# Autodesk Inventor assembly: Robot Assembly
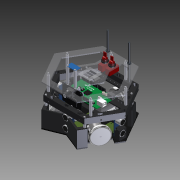
[picture p0: Inventor's stored thumbnail of the model, 180x180]
Saved by Autodesk Inventor 2015 (Build 190159000, 159)
## iProperties
Created: 2016-02-25
Part Number: Robot Assembly
Document SubType Name: Assembly
Designer: James Yelland
Author: James Yelland
## Documents named in this file (29)
- C:\Users\James Yelland\git\Design\Design\Models\Version 5\Robot Assembly.iam
- C:\Users\James Yelland\git\Design\Design\Models\Version 5\TSOP Array.ipt
- C:\Users\James Yelland\git\Design\Design\Models\Version 5\Bottom Plate.ipt
- C:\Users\James Yelland\git\Design\Design\Models\Version 5\Side Support.ipt
- C:\Users\James Yelland\git\Design\Design\Models\Version 5\Front Support.ipt
- C:\Users\James Yelland\git\Design\Design\Models\Version 5\Standoff 10.ipt
- C:\Users\James Yelland\git\Design\Design\Models\Common\Motor Mount Bracket.ipt
- C:\Users\James Yelland\git\Design\Design\Models\Common\Motor Mount Standoff.ipt
- C:\Users\James Yelland\git\Design\Design\Models\Common\Motor.ipt
- C:\Users\James Yelland\git\Design\Design\Models\Common\Wheel.ipt
- C:\Users\James Yelland\git\Design\Design\Models\Version 5\M3x10 Screw Nylon.ipt
- C:\Users\James Yelland\git\Design\Design\Models\Version 5\M3x20 Screw Nylon.ipt
- C:\Users\James Yelland\git\Design\Design\Models\Version 5\M3x6 Screw Nylon.ipt
- C:\Users\James Yelland\git\Design\Design\Models\Version 5\M3 Nut Steel.ipt
- C:\Users\James Yelland\git\Design\Design\Models\Version 5\M3x10 Screw Steel.ipt
- C:\Users\James Yelland\git\Design\Design\Models\Version 5\Standoff 40.ipt
- C:\Users\James Yelland\git\Design\Design\Models\Version 5\Top Plate.ipt
- C:\Users\James Yelland\git\Design\Design\Models\Version 5\Switch Nut.ipt
- C:\Users\James Yelland\git\Design\Design\Models\Version 5\Switch.ipt
- C:\Users\James Yelland\git\Design\Design\Models\Common\Compass.ipt
- C:\Users\James Yelland\git\Design\Design\Models\Version 5\Sonar Mount.ipt
- C:\Users\James Yelland\git\Design\Design\Models\Common\HC-SR04 Sonar.ipt
- C:\Users\James Yelland\git\Design\Design\Models\Version 5\M2x10 Screw Steel.ipt
- C:\Users\James Yelland\git\Design\Design\Models\Version 5\Light Sensors.ipt
- C:\Users\James Yelland\git\Design\Design\Models\Version 5\Rod.ipt
- C:\Users\James Yelland\git\Design\Design\Models\Version 5\Rod Nut.ipt
- C:\Users\James Yelland\git\Design\Design\Models\Imported Components\Pixy(CMUcam5)\Pixy(CMUcam5).iam
- C:\Users\James Yelland\git\Design\Design\Models\Version 5\M3 Nut Nylon.ipt
- C:\Users\James Yelland\git\Design\Design\Models\Common\ArduinoMEGA2560.ipt
## Components (125 placed, 28 different names)
1. TSOP Array:1 — Mate:22, Mate:23, Mate:24, Mate:67, Mate:68, Mate:69, Mate:70, Mate:71, Mate:72, Mate:73, Mate:74, Mate:236, Mate:291, Mate:292, Mate:295, Mate:296, Mate:297, Mate:298, Mate:299, Mate:302, Mate:303, Mate:304, Mate:305, Mate:306, Mate:310, Mate:312, Mate:313, Mate:314, Mate:316, Mate:317, Mate:318, Mate:320, Mate:321, Mate:322, Mate:323, Mate:325, Mate:352, Mate:353, Mate:354, Mate:355, Mate:360, Mate:361, Mate:362, Mate:363, Mate:364, Mate:365, Mate:366, Mate:367, Mate:368, Mate:369, Mate:370, Mate:371, Mate:372, Mate:373, Mate:374, Flush:6, Mate:390, Mate:392, Mate:394, Mate:396, Mate:398, Mate:400
2. Bottom Plate:1 — Mate:1, Mate:2, Mate:3, Mate:4, Mate:5, Mate:6, Mate:7, Mate:11, Mate:12, Mate:13, Mate:25, Mate:26, Mate:27, Mate:28, Mate:29, Mate:30, Mate:31, Mate:32, Mate:33, Mate:55, Mate:56, Mate:57, Mate:58, Mate:59, Mate:60, Mate:61, Mate:62, Mate:63, Mate:64, Mate:65, Mate:66, Mate:117, Mate:118, Mate:119, Mate:120, Mate:121, Mate:122, Mate:123, Mate:124, Mate:125, Mate:126, Mate:127, Mate:128, Mate:129, Mate:130, Mate:131, Mate:132, Mate:133, Mate:134, Mate:135, Mate:136, Mate:137, Mate:138, Mate:139, Mate:140, Mate:225, Mate:226, Mate:227, Mate:231, Mate:232, Mate:233, Mate:254, Mate:255, Mate:256, Mate:257, Mate:258, Mate:259, Mate:260, Mate:261, Mate:349, Mate:350, Mate:351
3. Side Support:1 — Mate:2, Mate:5, Mate:6, Mate:7, Mate:14, Mate:15
4. Side Support:2 — Mate:1, Mate:3, Mate:4, Mate:18, Mate:19
5. Front Support:1 — Mate:11, Mate:12, Mate:13, Mate:16, Mate:17, Mate:20, Mate:21, Mate:342, Mate:343, Mate:344
6. Standoff 10:1 — Mate:20, Mate:21, Mate:24
7. Standoff 10:2 — Mate:18, Mate:19
8. Standoff 10:3 — Mate:16, Mate:17, Mate:22, Mate:236
9. Standoff 10:4 — Mate:14, Mate:15, Mate:23
10. Motor Mount Bracket:1 — Mate:34, Mate:35, Mate:36, Mate:46, Mate:47, Mate:48, Mate:148, Mate:149, Mate:150, Mate:151
11. Motor Mount Standoff:1 — Mate:25, Mate:26, Mate:27, Mate:40, Mate:41, Mate:42
12. Motor:1 — Mate:43, Mate:44, Mate:45, Mate:52, Flush:1
13. Wheel:1 — Mate:52, Flush:1
14. Motor Mount Bracket:2 — Mate:37, Mate:38, Mate:39, Mate:49, Mate:50, Mate:51, Mate:141, Mate:143, Mate:146, Mate:147
15. Motor Mount Standoff:2 — Mate:28, Mate:29, Mate:30, Mate:34, Mate:35, Mate:36
16. Motor:2 — Mate:49, Mate:50, Mate:51, Mate:53, Flush:2
17. Wheel:2 — Mate:53, Flush:2
18. Motor Mount Bracket:3 — Mate:40, Mate:41, Mate:42, Mate:43, Mate:44, Mate:45, Mate:144, Mate:145, Mate:152, Mate:153
19. Motor Mount Standoff:3 — Mate:31, Mate:32, Mate:33, Mate:37, Mate:38, Mate:39
20. Motor:3 — Mate:46, Mate:47, Mate:48, Mate:54, Flush:3
21. Wheel:3 — Mate:54, Flush:3
22. M3x10 Screw Nylon:1 — Mate:59, Mate:60
23. M3x10 Screw Nylon:2 — Mate:61, Mate:62
24. M3x10 Screw Nylon:3 — Mate:63, Mate:66
25. M3x10 Screw Nylon:4 — Mate:64, Mate:65
26. M3x10 Screw Nylon:5 — Mate:55, Mate:56
27. M3x10 Screw Nylon:6 — Mate:57, Mate:58
28. M3x20 Screw Nylon:1 — Mate:70, Mate:74
29. M3x20 Screw Nylon:2 — Mate:69, Mate:72
30. M3x20 Screw Nylon:3 — Mate:68, Mate:71
31. M3x20 Screw Nylon:4 — Mate:67, Mate:73
32. M3 Nut Steel:1 — Mate:141, Mate:142
33. M3x10 Screw Steel:1 — Mate:117, Mate:139, Mate:142
34. M3 Nut Steel:2 — Mate:145, Mate:156
35. M3x10 Screw Steel:2 — Mate:119, Mate:136, Mate:158
36. M3 Nut Steel:3 — Mate:148, Mate:160
37. M3x10 Screw Steel:3 — Mate:120, Mate:137, Mate:157
38. M3 Nut Steel:4 — Mate:153, Mate:163
39. M3x10 Screw Steel:4 — Mate:121, Mate:129, Mate:160
40. M3 Nut Steel:5 — Mate:144, Mate:155
41. M3x10 Screw Steel:5 — Mate:118, Mate:140, Mate:159
42. M3 Nut Steel:6 — Mate:150, Mate:161
43. M3x10 Screw Steel:6 — Mate:122, Mate:130, Mate:162
44. M3 Nut Steel:7 — Mate:151, Mate:162
45. M3x10 Screw Steel:7 — Mate:124, Mate:131, Mate:161
46. M3 Nut Steel:8 — Mate:152, Mate:164
47. M3x10 Screw Steel:8 — Mate:126, Mate:133, Mate:164
48. M3 Nut Steel:9 — Mate:143, Mate:154
49. M3x10 Screw Steel:9 — Mate:123, Mate:138, Mate:154
50. M3 Nut Steel:10 — Mate:149, Mate:159
51. M3x10 Screw Steel:10 — Mate:125, Mate:134, Mate:156
52. M3 Nut Steel:11 — Mate:147, Mate:157
53. M3x10 Screw Steel:11 — Mate:127, Mate:132, Mate:163
54. M3 Nut Steel:12 — Mate:146, Mate:158
55. M3x10 Screw Steel:12 — Mate:128, Mate:135, Mate:155
56. Top Plate:1 — Mate:178, Mate:179, Flush:4, Flush:5, Mate:187, Mate:188, Mate:189, Mate:190, Mate:207, Mate:208, Mate:209, Mate:210, Mate:218, Mate:219, Mate:220, Mate:221, Mate:293, Mate:308, Mate:326, Mate:327, Mate:328, Mate:330, Mate:331, Mate:333, Mate:334, Mate:335, Mate:336, Mate:338, Mate:339, Mate:341, Mate:356, Mate:358
57. Switch Nut:1 — Mate:183, Mate:190
58. Switch:1 — Mate:178, Flush:4, Mate:183, Mate:187
59. Switch Nut:2 — Mate:181, Mate:189
60. Switch:2 — Mate:179, Flush:5, Mate:181, Mate:188
61. Standoff 40:5 — Mate:207, Mate:209, Mate:211, Mate:213
62. Standoff 40:6 — Mate:208, Mate:210, Mate:212
63. M3x10 Screw Nylon:11 — Mate:214, Mate:215
64. M3x10 Screw Nylon:12 — Mate:216, Mate:217
65. M3x10 Screw Nylon:13 — Mate:220, Mate:221
66. M3x10 Screw Nylon:14 — Mate:218, Mate:219
67. Compass:1 — Mate:211, Mate:212, Mate:213, Mate:214, Mate:215, Mate:216, Mate:217
68. Sonar Mount:1 — Mate:222, Mate:223, Mate:224, Mate:225, Mate:226, Mate:227
69. HC-SR04 Sonar:1 — Mate:222, Mate:223, Mate:224, Mate:265, Mate:266, Mate:267, Mate:268
70. Sonar Mount:3 — Mate:228, Mate:229, Mate:230, Mate:231, Mate:232, Mate:233
71. HC-SR04 Sonar:2 — Mate:228, Mate:229, Mate:230, Mate:262, Mate:263, Mate:264, Mate:269
72. M3x6 Screw Nylon:10 — Mate:258, Mate:259
73. M3x6 Screw Nylon:11 — Mate:260, Mate:261
74. M3x6 Screw Nylon:12 — Mate:256, Mate:257
75. M3x6 Screw Nylon:13 — Mate:254, Mate:255
76. M2x10 Screw Steel:1 — Mate:265, Mate:268
77. M2x10 Screw Steel:2 — Mate:264, Mate:269
78. M2x10 Screw Steel:3 — Mate:266, Mate:267
79. M2x10 Screw Steel:4 — Mate:262, Mate:263
80. M3x10 Screw Nylon:15 — Mate:331, Mate:339
81. M3x20 Screw Nylon:7 — Mate:312, Mate:321
82. Standoff 40:7 — Mate:291, Mate:292, Mate:293
83. M3x20 Screw Nylon:8 — Mate:313, Mate:322
84. M3x10 Screw Nylon:17 — Mate:333, Mate:341
85. M3x20 Screw Nylon:9 — Mate:314, Mate:323
86. Standoff 40:9 — Mate:298, Mate:302
87. M3x10 Screw Nylon:18 — Mate:328, Mate:336
88. Standoff 40:10 — Mate:296, Mate:305
89. M3x10 Screw Nylon:19 — Mate:327, Mate:334
90. M3x20 Screw Nylon:11 — Mate:316, Mate:325
91. Standoff 40:11 — Mate:297, Mate:304
92. M3x10 Screw Nylon:20 — Mate:326, Mate:335
93. M3x20 Screw Nylon:12 — Mate:317, Mate:318
94. Standoff 40:12 — Mate:299, Mate:303, Mate:308
95. M3x10 Screw Nylon:21 — Mate:330, Mate:338
96. M3x20 Screw Nylon:14 — Mate:310, Mate:320
97. Standoff 40:14 — Mate:295, Mate:306
98. HC-SR04 Sonar:3 — Mate:342, Mate:343, Mate:344, Mate:345, Mate:346, Mate:347, Mate:348
99. M2x10 Screw Steel:5 — Mate:347, Mate:348
100. M2x10 Screw Steel:6 — Mate:345, Mate:346
101. Light Sensors:1 — Mate:349, Mate:350, Mate:351
102. Rod:1 — Mate:352, Mate:355, Mate:359
103. Rod:2 — Mate:353, Mate:354, Mate:357
104. Rod Nut:1 — Mate:356, Mate:357
105. Rod Nut:2 — Mate:358, Mate:359
106. Pixy(CMUcam5):1 [sub-assembly] — Mate:360, Mate:361, Mate:362, Flush:6
107. Standoff 10:5 — Mate:363, Mate:364, Mate:377, Mate:391
108. Standoff 10:6 — Mate:365, Mate:366, Mate:401
109. Standoff 10:7 — Mate:367, Mate:368, Mate:376, Mate:395
110. Standoff 10:8 — Mate:369, Mate:370, Mate:375, Mate:393
111. Standoff 10:9 — Mate:371, Mate:372, Mate:397
112. Standoff 10:10 — Mate:373, Mate:374, Mate:399
113. M3x6 Screw Nylon:14 — Mate:378, Mate:379
114. M3x6 Screw Nylon:15 — Mate:382, Mate:383
115. M3x6 Screw Nylon:16 — Mate:386, Mate:387
116. M3x6 Screw Nylon:17 — Mate:388, Mate:389
117. M3x6 Screw Nylon:18 — Mate:384, Mate:385
118. M3x6 Screw Nylon:19 — Mate:380, Mate:381
119. M3 Nut Nylon:1 — Mate:400, Mate:401
120. M3 Nut Nylon:2 — Mate:398, Mate:399
121. M3 Nut Nylon:3 — Mate:396, Mate:397
122. M3 Nut Nylon:4 — Mate:394, Mate:395
123. M3 Nut Nylon:5 — Mate:392, Mate:393
124. M3 Nut Nylon:6 — Mate:390, Mate:391
125. -  -:1 — Mate:375, Mate:376, Mate:377, Mate:378, Mate:379, Mate:380, Mate:381, Mate:382, Mate:383, Mate:384, Mate:385, Mate:386, Mate:387, Mate:388, Mate:389
## Relationships (275: Mate 269, Flush 6)
- Mate:1: Bottom Plate:1 ↔ Side Support:2
- Mate:2: Bottom Plate:1 ↔ Side Support:1
- Mate:3: Bottom Plate:1 ↔ Side Support:2
- Mate:4: Bottom Plate:1 ↔ Side Support:2
- Mate:5: Bottom Plate:1 ↔ Side Support:1
- Mate:6: Bottom Plate:1 ↔ Side Support:1
- Mate:7: Bottom Plate:1 ↔ Side Support:1
- Mate:11: Bottom Plate:1 ↔ Front Support:1
- Mate:12: Bottom Plate:1 ↔ Front Support:1
- Mate:13: Bottom Plate:1 ↔ Front Support:1
- Mate:14: Side Support:1 ↔ Standoff 10:4
- Mate:15: Side Support:1 ↔ Standoff 10:4
- Mate:16: Front Support:1 ↔ Standoff 10:3
- Mate:17: Front Support:1 ↔ Standoff 10:3
- Mate:18: Side Support:2 ↔ Standoff 10:2
- Mate:19: Side Support:2 ↔ Standoff 10:2
- Mate:20: Front Support:1 ↔ Standoff 10:1
- Mate:21: Front Support:1 ↔ Standoff 10:1
- Mate:22: TSOP Array:1 ↔ Standoff 10:3
- Mate:23: TSOP Array:1 ↔ Standoff 10:4
- Mate:24: TSOP Array:1 ↔ Standoff 10:1
- Mate:25: Bottom Plate:1 ↔ Motor Mount Standoff:1
- Mate:26: Bottom Plate:1 ↔ Motor Mount Standoff:1
- Mate:27: Bottom Plate:1 ↔ Motor Mount Standoff:1
- Mate:28: Bottom Plate:1 ↔ Motor Mount Standoff:2
- Mate:29: Bottom Plate:1 ↔ Motor Mount Standoff:2
- Mate:30: Bottom Plate:1 ↔ Motor Mount Standoff:2
- Mate:31: Bottom Plate:1 ↔ Motor Mount Standoff:3
- Mate:32: Bottom Plate:1 ↔ Motor Mount Standoff:3
- Mate:33: Bottom Plate:1 ↔ Motor Mount Standoff:3
- Mate:34: Motor Mount Bracket:1 ↔ Motor Mount Standoff:2
- Mate:35: Motor Mount Bracket:1 ↔ Motor Mount Standoff:2
- Mate:36: Motor Mount Bracket:1 ↔ Motor Mount Standoff:2
- Mate:37: Motor Mount Bracket:2 ↔ Motor Mount Standoff:3
- Mate:38: Motor Mount Bracket:2 ↔ Motor Mount Standoff:3
- Mate:39: Motor Mount Bracket:2 ↔ Motor Mount Standoff:3
- Mate:40: Motor Mount Standoff:1 ↔ Motor Mount Bracket:3
- Mate:41: Motor Mount Standoff:1 ↔ Motor Mount Bracket:3
- Mate:42: Motor Mount Standoff:1 ↔ Motor Mount Bracket:3
- Mate:43: Motor:1 ↔ Motor Mount Bracket:3
- Mate:44: Motor:1 ↔ Motor Mount Bracket:3
- Mate:45: Motor:1 ↔ Motor Mount Bracket:3
- Mate:46: Motor Mount Bracket:1 ↔ Motor:3
- Mate:47: Motor Mount Bracket:1 ↔ Motor:3
- Mate:48: Motor Mount Bracket:1 ↔ Motor:3
- Mate:49: Motor Mount Bracket:2 ↔ Motor:2
- Mate:50: Motor Mount Bracket:2 ↔ Motor:2
- Mate:51: Motor Mount Bracket:2 ↔ Motor:2
- Mate:52: Motor:1 ↔ Wheel:1
- Flush:1: Motor:1 ↔ Wheel:1
- Mate:53: Motor:2 ↔ Wheel:2
- Flush:2: Motor:2 ↔ Wheel:2
- Mate:54: Motor:3 ↔ Wheel:3
- Flush:3: Motor:3 ↔ Wheel:3
- Mate:55: Bottom Plate:1 ↔ M3x10 Screw Nylon:5
- Mate:56: Bottom Plate:1 ↔ M3x10 Screw Nylon:5
- Mate:57: Bottom Plate:1 ↔ M3x10 Screw Nylon:6
- Mate:58: Bottom Plate:1 ↔ M3x10 Screw Nylon:6
- Mate:59: Bottom Plate:1 ↔ M3x10 Screw Nylon:1
- Mate:60: Bottom Plate:1 ↔ M3x10 Screw Nylon:1
- Mate:61: Bottom Plate:1 ↔ M3x10 Screw Nylon:2
- Mate:62: Bottom Plate:1 ↔ M3x10 Screw Nylon:2
- Mate:63: Bottom Plate:1 ↔ M3x10 Screw Nylon:3
- Mate:64: Bottom Plate:1 ↔ M3x10 Screw Nylon:4
- Mate:65: Bottom Plate:1 ↔ M3x10 Screw Nylon:4
- Mate:66: Bottom Plate:1 ↔ M3x10 Screw Nylon:3
- Mate:67: TSOP Array:1 ↔ M3x20 Screw Nylon:4
- Mate:68: TSOP Array:1 ↔ M3x20 Screw Nylon:3
- Mate:69: TSOP Array:1 ↔ M3x20 Screw Nylon:2
- Mate:70: TSOP Array:1 ↔ M3x20 Screw Nylon:1
- Mate:71: TSOP Array:1 ↔ M3x20 Screw Nylon:3
- Mate:72: TSOP Array:1 ↔ M3x20 Screw Nylon:2
- Mate:73: TSOP Array:1 ↔ M3x20 Screw Nylon:4
- Mate:74: TSOP Array:1 ↔ M3x20 Screw Nylon:1
- Mate:117: Bottom Plate:1 ↔ M3x10 Screw Steel:1
- Mate:118: Bottom Plate:1 ↔ M3x10 Screw Steel:5
- Mate:119: Bottom Plate:1 ↔ M3x10 Screw Steel:2
- Mate:120: Bottom Plate:1 ↔ M3x10 Screw Steel:3
- Mate:121: Bottom Plate:1 ↔ M3x10 Screw Steel:4
- Mate:122: Bottom Plate:1 ↔ M3x10 Screw Steel:6
- Mate:123: Bottom Plate:1 ↔ M3x10 Screw Steel:9
- Mate:124: Bottom Plate:1 ↔ M3x10 Screw Steel:7
- Mate:125: Bottom Plate:1 ↔ M3x10 Screw Steel:10
- Mate:126: Bottom Plate:1 ↔ M3x10 Screw Steel:8
- Mate:127: Bottom Plate:1 ↔ M3x10 Screw Steel:11
- Mate:128: Bottom Plate:1 ↔ M3x10 Screw Steel:12
- Mate:129: Bottom Plate:1 ↔ M3x10 Screw Steel:4
- Mate:130: Bottom Plate:1 ↔ M3x10 Screw Steel:6
- Mate:131: Bottom Plate:1 ↔ M3x10 Screw Steel:7
- Mate:132: Bottom Plate:1 ↔ M3x10 Screw Steel:11
- Mate:133: Bottom Plate:1 ↔ M3x10 Screw Steel:8
- Mate:134: Bottom Plate:1 ↔ M3x10 Screw Steel:10
- Mate:135: Bottom Plate:1 ↔ M3x10 Screw Steel:12
- Mate:136: Bottom Plate:1 ↔ M3x10 Screw Steel:2
- Mate:137: Bottom Plate:1 ↔ M3x10 Screw Steel:3
- Mate:138: Bottom Plate:1 ↔ M3x10 Screw Steel:9
- Mate:139: Bottom Plate:1 ↔ M3x10 Screw Steel:1
- Mate:140: Bottom Plate:1 ↔ M3x10 Screw Steel:5
- Mate:141: Motor Mount Bracket:2 ↔ M3 Nut Steel:1
- Mate:142: M3 Nut Steel:1 ↔ M3x10 Screw Steel:1
- Mate:143: Motor Mount Bracket:2 ↔ M3 Nut Steel:9
- Mate:144: Motor Mount Bracket:3 ↔ M3 Nut Steel:5
- Mate:145: Motor Mount Bracket:3 ↔ M3 Nut Steel:2
- Mate:146: Motor Mount Bracket:2 ↔ M3 Nut Steel:12
- Mate:147: Motor Mount Bracket:2 ↔ M3 Nut Steel:11
- Mate:148: Motor Mount Bracket:1 ↔ M3 Nut Steel:3
- Mate:149: Motor Mount Bracket:1 ↔ M3 Nut Steel:10
- Mate:150: Motor Mount Bracket:1 ↔ M3 Nut Steel:6
- Mate:151: Motor Mount Bracket:1 ↔ M3 Nut Steel:7
- Mate:152: Motor Mount Bracket:3 ↔ M3 Nut Steel:8
- Mate:153: Motor Mount Bracket:3 ↔ M3 Nut Steel:4
- Mate:154: M3 Nut Steel:9 ↔ M3x10 Screw Steel:9
- Mate:155: M3 Nut Steel:5 ↔ M3x10 Screw Steel:12
- Mate:156: M3 Nut Steel:2 ↔ M3x10 Screw Steel:10
- Mate:157: M3x10 Screw Steel:3 ↔ M3 Nut Steel:11
- Mate:158: M3x10 Screw Steel:2 ↔ M3 Nut Steel:12
- Mate:159: M3x10 Screw Steel:5 ↔ M3 Nut Steel:10
- Mate:160: M3 Nut Steel:3 ↔ M3x10 Screw Steel:4
- Mate:161: M3 Nut Steel:6 ↔ M3x10 Screw Steel:7
- Mate:162: M3x10 Screw Steel:6 ↔ M3 Nut Steel:7
- Mate:163: M3 Nut Steel:4 ↔ M3x10 Screw Steel:11
- Mate:164: M3 Nut Steel:8 ↔ M3x10 Screw Steel:8
- Mate:178: Top Plate:1 ↔ Switch:1
- Mate:179: Top Plate:1 ↔ Switch:2
- Flush:4 (4 mm): Top Plate:1 ↔ Switch:1
- Flush:5 (4 mm): Top Plate:1 ↔ Switch:2
- Mate:181: Switch Nut:2 ↔ Switch:2
- Mate:183: Switch Nut:1 ↔ Switch:1
- Mate:187: Top Plate:1 ↔ Switch:1
- Mate:188: Top Plate:1 ↔ Switch:2
- Mate:189: Top Plate:1 ↔ Switch Nut:2
- Mate:190: Top Plate:1 ↔ Switch Nut:1
- Mate:207: Top Plate:1 ↔ Standoff 40:5
- Mate:208: Top Plate:1 ↔ Standoff 40:6
- Mate:209: Top Plate:1 ↔ Standoff 40:5
- Mate:210: Top Plate:1 ↔ Standoff 40:6
- Mate:211: Standoff 40:5 ↔ Compass:1
- Mate:212: Standoff 40:6 ↔ Compass:1
- Mate:213: Standoff 40:5 ↔ Compass:1
- Mate:214: M3x10 Screw Nylon:11 ↔ Compass:1
- Mate:215: M3x10 Screw Nylon:11 ↔ Compass:1
- Mate:216: M3x10 Screw Nylon:12 ↔ Compass:1
- Mate:217: M3x10 Screw Nylon:12 ↔ Compass:1
- Mate:218: Top Plate:1 ↔ M3x10 Screw Nylon:14
- Mate:219: Top Plate:1 ↔ M3x10 Screw Nylon:14
- Mate:220: Top Plate:1 ↔ M3x10 Screw Nylon:13
- Mate:221: Top Plate:1 ↔ M3x10 Screw Nylon:13
- Mate:222: Sonar Mount:1 ↔ HC-SR04 Sonar:1
- Mate:223: Sonar Mount:1 ↔ HC-SR04 Sonar:1
- Mate:224: Sonar Mount:1 ↔ HC-SR04 Sonar:1
- Mate:225: Bottom Plate:1 ↔ Sonar Mount:1
- Mate:226: Bottom Plate:1 ↔ Sonar Mount:1
- Mate:227: Bottom Plate:1 ↔ Sonar Mount:1
- Mate:228: Sonar Mount:3 ↔ HC-SR04 Sonar:2
- Mate:229: Sonar Mount:3 ↔ HC-SR04 Sonar:2
- Mate:230: Sonar Mount:3 ↔ HC-SR04 Sonar:2
- Mate:231: Bottom Plate:1 ↔ Sonar Mount:3
- Mate:232: Bottom Plate:1 ↔ Sonar Mount:3
- Mate:233: Bottom Plate:1 ↔ Sonar Mount:3
- Mate:236: TSOP Array:1 ↔ Standoff 10:3
- Mate:254: Bottom Plate:1 ↔ M3x6 Screw Nylon:13
- Mate:255: Bottom Plate:1 ↔ M3x6 Screw Nylon:13
- Mate:256: Bottom Plate:1 ↔ M3x6 Screw Nylon:12
- Mate:257: Bottom Plate:1 ↔ M3x6 Screw Nylon:12
- Mate:258: Bottom Plate:1 ↔ M3x6 Screw Nylon:10
- Mate:259: Bottom Plate:1 ↔ M3x6 Screw Nylon:10
- Mate:260: Bottom Plate:1 ↔ M3x6 Screw Nylon:11
- Mate:261: Bottom Plate:1 ↔ M3x6 Screw Nylon:11
- Mate:262: HC-SR04 Sonar:2 ↔ M2x10 Screw Steel:4
- Mate:263: HC-SR04 Sonar:2 ↔ M2x10 Screw Steel:4
- Mate:264: HC-SR04 Sonar:2 ↔ M2x10 Screw Steel:2
- Mate:265: HC-SR04 Sonar:1 ↔ M2x10 Screw Steel:1
- Mate:266: HC-SR04 Sonar:1 ↔ M2x10 Screw Steel:3
- Mate:267: HC-SR04 Sonar:1 ↔ M2x10 Screw Steel:3
- Mate:268: HC-SR04 Sonar:1 ↔ M2x10 Screw Steel:1
- Mate:269: HC-SR04 Sonar:2 ↔ M2x10 Screw Steel:2
- Mate:291: TSOP Array:1 ↔ Standoff 40:7
- Mate:292: TSOP Array:1 ↔ Standoff 40:7
- Mate:293: Top Plate:1 ↔ Standoff 40:7
- Mate:295: TSOP Array:1 ↔ Standoff 40:14
- Mate:296: TSOP Array:1 ↔ Standoff 40:10
- Mate:297: TSOP Array:1 ↔ Standoff 40:11
- Mate:298: TSOP Array:1 ↔ Standoff 40:9
- Mate:299: TSOP Array:1 ↔ Standoff 40:12
- Mate:302: TSOP Array:1 ↔ Standoff 40:9
- Mate:303: TSOP Array:1 ↔ Standoff 40:12
- Mate:304: TSOP Array:1 ↔ Standoff 40:11
- Mate:305: TSOP Array:1 ↔ Standoff 40:10
- Mate:306: TSOP Array:1 ↔ Standoff 40:14
- Mate:308: Top Plate:1 ↔ Standoff 40:12
- Mate:310: TSOP Array:1 ↔ M3x20 Screw Nylon:14
- Mate:312: TSOP Array:1 ↔ M3x20 Screw Nylon:7
- Mate:313: TSOP Array:1 ↔ M3x20 Screw Nylon:8
- Mate:314: TSOP Array:1 ↔ M3x20 Screw Nylon:9
- Mate:316: TSOP Array:1 ↔ M3x20 Screw Nylon:11
- Mate:317: TSOP Array:1 ↔ M3x20 Screw Nylon:12
- Mate:318: TSOP Array:1 ↔ M3x20 Screw Nylon:12
- Mate:320: TSOP Array:1 ↔ M3x20 Screw Nylon:14
- Mate:321: TSOP Array:1 ↔ M3x20 Screw Nylon:7
- Mate:322: TSOP Array:1 ↔ M3x20 Screw Nylon:8
- Mate:323: TSOP Array:1 ↔ M3x20 Screw Nylon:9
- Mate:325: TSOP Array:1 ↔ M3x20 Screw Nylon:11
- Mate:326: Top Plate:1 ↔ M3x10 Screw Nylon:20
- Mate:327: Top Plate:1 ↔ M3x10 Screw Nylon:19
- Mate:328: Top Plate:1 ↔ M3x10 Screw Nylon:18
- Mate:330: Top Plate:1 ↔ M3x10 Screw Nylon:21
- Mate:331: Top Plate:1 ↔ M3x10 Screw Nylon:15
- Mate:333: Top Plate:1 ↔ M3x10 Screw Nylon:17
- Mate:334: Top Plate:1 ↔ M3x10 Screw Nylon:19
- Mate:335: Top Plate:1 ↔ M3x10 Screw Nylon:20
- Mate:336: Top Plate:1 ↔ M3x10 Screw Nylon:18
- Mate:338: Top Plate:1 ↔ M3x10 Screw Nylon:21
- Mate:339: Top Plate:1 ↔ M3x10 Screw Nylon:15
- Mate:341: Top Plate:1 ↔ M3x10 Screw Nylon:17
- Mate:342: Front Support:1 ↔ HC-SR04 Sonar:3
- Mate:343: Front Support:1 ↔ HC-SR04 Sonar:3
- Mate:344: Front Support:1 ↔ HC-SR04 Sonar:3
- Mate:345: HC-SR04 Sonar:3 ↔ M2x10 Screw Steel:6
- Mate:346: HC-SR04 Sonar:3 ↔ M2x10 Screw Steel:6
- Mate:347: HC-SR04 Sonar:3 ↔ M2x10 Screw Steel:5
- Mate:348: HC-SR04 Sonar:3 ↔ M2x10 Screw Steel:5
- Mate:349 (5 mm): Bottom Plate:1 ↔ Light Sensors:1
- Mate:350: Bottom Plate:1 ↔ Light Sensors:1
- Mate:351: Bottom Plate:1 ↔ Light Sensors:1
- Mate:352: TSOP Array:1 ↔ Rod:1
- Mate:353: TSOP Array:1 ↔ Rod:2
- Mate:354: TSOP Array:1 ↔ Rod:2
- Mate:355: TSOP Array:1 ↔ Rod:1
- Mate:356: Top Plate:1 ↔ Rod Nut:1
- Mate:357: Rod:2 ↔ Rod Nut:1
- Mate:358: Top Plate:1 ↔ Rod Nut:2
- Mate:359: Rod:1 ↔ Rod Nut:2
- Mate:360 (10 mm): TSOP Array:1 ↔ Pixy(CMUcam5):1
- Mate:361: TSOP Array:1 ↔ Pixy(CMUcam5):1
- Mate:362: TSOP Array:1 ↔ Pixy(CMUcam5):1
- Mate:363: TSOP Array:1 ↔ Standoff 10:5
- Mate:364: TSOP Array:1 ↔ Standoff 10:5
- Mate:365: TSOP Array:1 ↔ Standoff 10:6
- Mate:366: TSOP Array:1 ↔ Standoff 10:6
- Mate:367: TSOP Array:1 ↔ Standoff 10:7
- Mate:368: TSOP Array:1 ↔ Standoff 10:7
- Mate:369: TSOP Array:1 ↔ Standoff 10:8
- Mate:370: TSOP Array:1 ↔ Standoff 10:8
- Mate:371: TSOP Array:1 ↔ Standoff 10:9
- Mate:372: TSOP Array:1 ↔ Standoff 10:9
- Mate:373: TSOP Array:1 ↔ Standoff 10:10
- Mate:374: TSOP Array:1 ↔ Standoff 10:10
- Mate:375: Standoff 10:8 ↔ -  -:1
- Mate:376: Standoff 10:7 ↔ -  -:1
- Mate:377: Standoff 10:5 ↔ -  -:1
- Mate:378: M3x6 Screw Nylon:14 ↔ -  -:1
- Mate:379: M3x6 Screw Nylon:14 ↔ -  -:1
- Mate:380: M3x6 Screw Nylon:19 ↔ -  -:1
- Mate:381: M3x6 Screw Nylon:19 ↔ -  -:1
- Mate:382: M3x6 Screw Nylon:15 ↔ -  -:1
- Mate:383: M3x6 Screw Nylon:15 ↔ -  -:1
- Mate:384: M3x6 Screw Nylon:18 ↔ -  -:1
- Mate:385: M3x6 Screw Nylon:18 ↔ -  -:1
- Mate:386: M3x6 Screw Nylon:16 ↔ -  -:1
- Mate:387: M3x6 Screw Nylon:16 ↔ -  -:1
- Mate:388: M3x6 Screw Nylon:17 ↔ -  -:1
- Mate:389: M3x6 Screw Nylon:17 ↔ -  -:1
- Flush:6 (3 mm): TSOP Array:1 ↔ Pixy(CMUcam5):1
- Mate:390: TSOP Array:1 ↔ M3 Nut Nylon:6
- Mate:391: Standoff 10:5 ↔ M3 Nut Nylon:6
- Mate:392: TSOP Array:1 ↔ M3 Nut Nylon:5
- Mate:393: Standoff 10:8 ↔ M3 Nut Nylon:5
- Mate:394: TSOP Array:1 ↔ M3 Nut Nylon:4
- Mate:395: Standoff 10:7 ↔ M3 Nut Nylon:4
- Mate:396: TSOP Array:1 ↔ M3 Nut Nylon:3
- Mate:397: Standoff 10:9 ↔ M3 Nut Nylon:3
- Mate:398: TSOP Array:1 ↔ M3 Nut Nylon:2
- Mate:399: Standoff 10:10 ↔ M3 Nut Nylon:2
- Mate:400: TSOP Array:1 ↔ M3 Nut Nylon:1
- Mate:401: Standoff 10:6 ↔ M3 Nut Nylon:1
